# Autodesk Inventor assembly: Assembly_Sensor2DoF
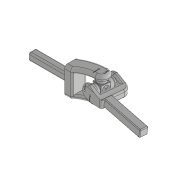
[picture p0: Inventor's stored thumbnail of the model, 180x180]
Saved by Autodesk Inventor 2020 (Build 240168000, 168)
## iProperties
Created: 2021-04-25
Part Number: Assembly_Sensor2DoF
Document SubType Name: Assembly
Designer: deox
Author: deox
## Documents named in this file (4)
- C:\Users\deox\Desktop\TCC\Inventor Files\2DoF Sensor\Assembly_Sensor2DoF.iam
- C:\Users\deox\Desktop\TCC\Inventor Files\2DoF Sensor\Cross.ipt
- C:\Users\deox\Desktop\TCC\Inventor Files\2DoF Sensor\Part1.ipt
- C:\Users\deox\Desktop\TCC\Inventor Files\2DoF Sensor\Part2.ipt
## Components (3 placed, 3 different names)
1. Cross:1 — Mate:1, Mate:2, Mate:3, Mate:4
2. Part1:1 — Mate:1, Mate:4
3. Part2:1 — Mate:2, Mate:3
## Relationships (4: Mate 4)
- Mate:1: Cross:1 ↔ Part1:1
- Mate:2: Cross:1 ↔ Part2:1
- Mate:3: Cross:1 ↔ Part2:1
- Mate:4: Cross:1 ↔ Part1:1
